# Autodesk Inventor assembly: 276-2158
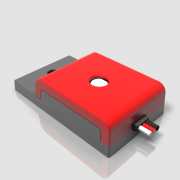
[picture p0: Inventor's stored thumbnail of the model, 180x180]
Saved by Autodesk Inventor 2015 SP1 (Build 190201100, 201)
## iProperties
Category: Sensors
Company: Super Sonic Sparks, Team 24
Part Number: 276-2158
Document SubType Name: Assembly
Designer: Jordan Kiesel
Mass: 11.793 g
Surface Area: 84.774 cm^2
Volume: 5.48885 cm^3
Density: 2.14854 g/cm^3
Catalog Web Link: vexrobotics.com/276-2158.html
Description: Uses a photocell that allows your robot to detect and react to light.
Vendor: VEX Robotics, Inc.
Translation Standard: STEP AP203
FileName: Light Sensor.iam
PreProcessor: SolidWorks 2006052
PostProcessor: Build: 239, Release: 2011 RTM - Date: Wed 02/17/2010
Sent Units: inch
Uncertainty: 1e-05
Author: Jordan Kiesel
Title: Light Sensor
Comments: The light sensor uses a photocell that allows your robot to detect and react to light. With the light sensor, you can program a whole new range of capabilities to your robot. A Programming Kit is needed to change the program in the VEX Controller. ▷ Analog input of light levels. ▷ Usable range of 0 to 6 feet. ▷ Find dark or bright areas. ▷ Create more autonomous function.
## Documents named in this file (6)
- C:\Users\Jordan\Documents\Robotics\VEX\CAD\2015 BNS CAD Library (beta)\Sensors\Light Sensor.iam
- C:\Users\Jordan\Documents\Robotics\VEX\CAD\2015 BNS CAD Library (beta)\Sensors\Reference Parts\Light Sensor\Bottom.ipt
- C:\Users\Jordan\Documents\Robotics\VEX\CAD\2015 BNS CAD Library (beta)\Sensors\Reference Parts\Sensors\Wire Sleeve.ipt
- C:\Users\Jordan\Documents\Robotics\VEX\CAD\2015 BNS CAD Library (beta)\Sensors\Reference Parts\Light Sensor\Top.ipt
- C:\Users\Jordan\Documents\Robotics\VEX\CAD\2015 BNS CAD Library (beta)\Sensors\Reference Parts\Light Sensor\PCB.ipt
- C:\Users\Jordan\Documents\Robotics\VEX\CAD\2015 BNS CAD Library (beta)\Sensors\Reference Parts\Sensors\3-Wire Black-Red-White Cable, Cut.ipt
## Components (5 placed, 5 different names)
1. Bottom:1 — Insert:1, Mate:1, Mate:2, Insert:2, Insert:3
2. Wire Sleeve:1 — Tangent:2, Tangent:3, Tangent:4, Angle:1
3. Top:1 — Insert:2, Insert:3
4. PCB:1 — Insert:1, Mate:1, Mate:2
5. 3-Wire Black-Red-White Cable, Cut:1 — Tangent:2, Tangent:3, Tangent:4, Angle:1
## Relationships (9: Tangent 3, Insert 3, Mate 2, Angle 1)
- Tangent:2 (0.4064 mm): Wire Sleeve:1 ↔ 3-Wire Black-Red-White Cable, Cut:1
- Tangent:3 (0.4064 mm): Wire Sleeve:1 ↔ 3-Wire Black-Red-White Cable, Cut:1
- Tangent:4 (0.2286 mm): Wire Sleeve:1 ↔ 3-Wire Black-Red-White Cable, Cut:1
- Insert:1: Bottom:1 ↔ PCB:1
- Mate:1: Bottom:1 ↔ PCB:1
- Mate:2: Bottom:1 ↔ PCB:1
- Angle:1 (0 deg): Wire Sleeve:1 ↔ 3-Wire Black-Red-White Cable, Cut:1
- Insert:2: Bottom:1 ↔ Top:1
- Insert:3: Bottom:1 ↔ Top:1
